# Autodesk Inventor assembly: BUMP_000_Bumpers
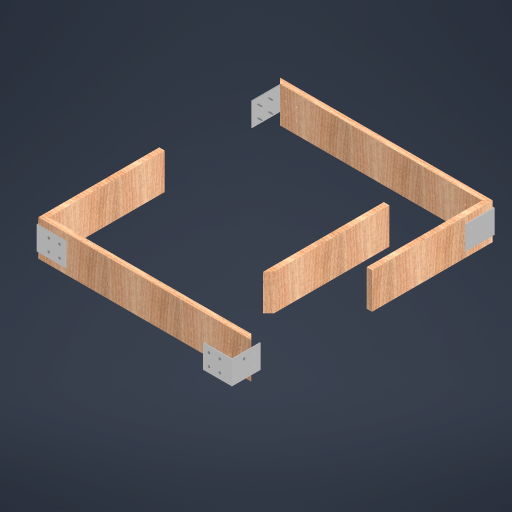
[picture p0: Inventor's stored thumbnail of the model, 512x512]
Saved by Autodesk Inventor 2024.2 (Build 282272000, 272)
## iProperties
Created: 2024-08-06
Part Number: BUMP_000_Bumpers
Document SubType Name: Assembly
Designer: Bryan
Author: Bryan
## Documents named in this file (5)
- C:\Users\bobsb\OneDrive\Documents\GitHub\1622-2024-Summer-CAD-A-Thon\Bumper\BUMP_000_Bumpers.iam
- C:\Users\bobsb\OneDrive\Documents\GitHub\1622-2024-Summer-CAD-A-Thon\Bumper\BUMP_001_Wood1.ipt
- C:\Users\bobsb\OneDrive\Documents\GitHub\1622-2024-Summer-CAD-A-Thon\Bumper\BUMP_002_Wood2.ipt
- C:\Users\bobsb\OneDrive\Documents\GitHub\1622-2024-Summer-CAD-A-Thon\COTS Library\Stucture\COTS_88805K219_Architectural 6063 Aluminum 90 Degree Angle.ipt
- C:\Users\bobsb\OneDrive\Documents\GitHub\1622-2024-Summer-CAD-A-Thon\COTS Library\Fasteners\Wood Screws\COTS_BumperWoodScrew_90031A197_Phillips Flat Head Screws for Wood.ipt
## Components (30 placed, 4 different names)
1. BUMP_001_Wood1:1 — Mate:5, Mate:6, Flush:3, Mate:12, Mate:13
2. BUMP_002_Wood2:1 — Flush:2, Mate:5, Mate:6, Flush:3, Mate:14
3. BUMP_001_Wood1:2 — Mate:1, Flush:1, Mate:2, Flush:2, Mate:7, Mate:9, Mate:27
4. BUMP_002_Wood2:2 — Mate:1, Flush:1, Mate:2, Mate:8
5. COTS_88805K219_Architectural 6063 Aluminum 90 Degree Angle:1 — Mate:7, Mate:8, Mate:19, Mate:20, Mate:21, Mate:22
6. COTS_88805K219_Architectural 6063 Aluminum 90 Degree Angle:2 — Mate:9, Mate:23, Mate:24, Mate:25, Mate:26
7. COTS_88805K219_Architectural 6063 Aluminum 90 Degree Angle:3 — Mate:13, Mate:14
8. COTS_88805K219_Architectural 6063 Aluminum 90 Degree Angle:4 — Mate:12, Mate:15, Mate:16, Mate:17, Mate:18
9. COTS_BumperWoodScrew_90031A197_Phillips Flat Head Screws for Wood:21 — Mate:25, Mate:26
10. BUMP_002_Wood2:3
11. COTS_BumperWoodScrew_90031A197_Phillips Flat Head Screws for Wood:1 — Mate:15, Mate:16
12. COTS_BumperWoodScrew_90031A197_Phillips Flat Head Screws for Wood:2
13. COTS_BumperWoodScrew_90031A197_Phillips Flat Head Screws for Wood:3
14. COTS_BumperWoodScrew_90031A197_Phillips Flat Head Screws for Wood:4
15. COTS_BumperWoodScrew_90031A197_Phillips Flat Head Screws for Wood:5 — Mate:17, Mate:18
16. COTS_BumperWoodScrew_90031A197_Phillips Flat Head Screws for Wood:6
17. COTS_BumperWoodScrew_90031A197_Phillips Flat Head Screws for Wood:7
18. COTS_BumperWoodScrew_90031A197_Phillips Flat Head Screws for Wood:8
19. COTS_BumperWoodScrew_90031A197_Phillips Flat Head Screws for Wood:9 — Mate:19, Mate:20
20. COTS_BumperWoodScrew_90031A197_Phillips Flat Head Screws for Wood:10
21. COTS_BumperWoodScrew_90031A197_Phillips Flat Head Screws for Wood:11
22. COTS_BumperWoodScrew_90031A197_Phillips Flat Head Screws for Wood:12
23. COTS_BumperWoodScrew_90031A197_Phillips Flat Head Screws for Wood:13 — Mate:21, Mate:22
24. COTS_BumperWoodScrew_90031A197_Phillips Flat Head Screws for Wood:14
25. COTS_BumperWoodScrew_90031A197_Phillips Flat Head Screws for Wood:15
26. COTS_BumperWoodScrew_90031A197_Phillips Flat Head Screws for Wood:16
27. COTS_BumperWoodScrew_90031A197_Phillips Flat Head Screws for Wood:17 — Mate:23, Mate:24
28. COTS_BumperWoodScrew_90031A197_Phillips Flat Head Screws for Wood:18
29. COTS_BumperWoodScrew_90031A197_Phillips Flat Head Screws for Wood:19 — Mate:27
30. COTS_BumperWoodScrew_90031A197_Phillips Flat Head Screws for Wood:20
## Component patterns: (4 elements, first: COTS_BumperWoodScrew_90031A197_Phillips Flat Head Screws for Wood:1), (4 elements, first: COTS_BumperWoodScrew_90031A197_Phillips Flat Head Screws for Wood:5), (4 elements, first: COTS_BumperWoodScrew_90031A197_Phillips Flat Head Screws for Wood:9), (4 elements, first: COTS_BumperWoodScrew_90031A197_Phillips Flat Head Screws for Wood:13), (4 elements, first: COTS_BumperWoodScrew_90031A197_Phillips Flat Head Screws for Wood:17)
## Relationships (26: Mate 23, Flush 3)
- Mate:1: BUMP_001_Wood1:2 ↔ BUMP_002_Wood2:2
- Flush:1: BUMP_001_Wood1:2 ↔ BUMP_002_Wood2:2
- Mate:2: BUMP_001_Wood1:2 ↔ BUMP_002_Wood2:2
- Flush:2: BUMP_002_Wood2:1 ↔ BUMP_001_Wood1:2
- Mate:5: BUMP_001_Wood1:1 ↔ BUMP_002_Wood2:1
- Mate:6: BUMP_001_Wood1:1 ↔ BUMP_002_Wood2:1
- Flush:3: BUMP_001_Wood1:1 ↔ BUMP_002_Wood2:1
- Mate:7: BUMP_001_Wood1:2 ↔ COTS_88805K219_Architectural 6063 Aluminum 90 Degree Angle:1
- Mate:8: BUMP_002_Wood2:2 ↔ COTS_88805K219_Architectural 6063 Aluminum 90 Degree Angle:1
- Mate:9: BUMP_001_Wood1:2 ↔ COTS_88805K219_Architectural 6063 Aluminum 90 Degree Angle:2
- Mate:12: BUMP_001_Wood1:1 ↔ COTS_88805K219_Architectural 6063 Aluminum 90 Degree Angle:4
- Mate:13: BUMP_001_Wood1:1 ↔ COTS_88805K219_Architectural 6063 Aluminum 90 Degree Angle:3
- Mate:14: BUMP_002_Wood2:1 ↔ COTS_88805K219_Architectural 6063 Aluminum 90 Degree Angle:3
- Mate:15: COTS_88805K219_Architectural 6063 Aluminum 90 Degree Angle:4 ↔ COTS_BumperWoodScrew_90031A197_Phillips Flat Head Screws for Wood:1
- Mate:16: COTS_88805K219_Architectural 6063 Aluminum 90 Degree Angle:4 ↔ COTS_BumperWoodScrew_90031A197_Phillips Flat Head Screws for Wood:1
- Mate:17: COTS_88805K219_Architectural 6063 Aluminum 90 Degree Angle:4 ↔ COTS_BumperWoodScrew_90031A197_Phillips Flat Head Screws for Wood:5
- Mate:18: COTS_88805K219_Architectural 6063 Aluminum 90 Degree Angle:4 ↔ COTS_BumperWoodScrew_90031A197_Phillips Flat Head Screws for Wood:5
- Mate:19: COTS_88805K219_Architectural 6063 Aluminum 90 Degree Angle:1 ↔ COTS_BumperWoodScrew_90031A197_Phillips Flat Head Screws for Wood:9
- Mate:20: COTS_88805K219_Architectural 6063 Aluminum 90 Degree Angle:1 ↔ COTS_BumperWoodScrew_90031A197_Phillips Flat Head Screws for Wood:9
- Mate:21: COTS_88805K219_Architectural 6063 Aluminum 90 Degree Angle:1 ↔ COTS_BumperWoodScrew_90031A197_Phillips Flat Head Screws for Wood:13
- Mate:22: COTS_88805K219_Architectural 6063 Aluminum 90 Degree Angle:1 ↔ COTS_BumperWoodScrew_90031A197_Phillips Flat Head Screws for Wood:13
- Mate:23: COTS_88805K219_Architectural 6063 Aluminum 90 Degree Angle:2 ↔ COTS_BumperWoodScrew_90031A197_Phillips Flat Head Screws for Wood:17
- Mate:24: COTS_88805K219_Architectural 6063 Aluminum 90 Degree Angle:2 ↔ COTS_BumperWoodScrew_90031A197_Phillips Flat Head Screws for Wood:17
- Mate:25: COTS_88805K219_Architectural 6063 Aluminum 90 Degree Angle:2 ↔ COTS_BumperWoodScrew_90031A197_Phillips Flat Head Screws for Wood:21
- Mate:26: COTS_88805K219_Architectural 6063 Aluminum 90 Degree Angle:2 ↔ COTS_BumperWoodScrew_90031A197_Phillips Flat Head Screws for Wood:21
- Mate:27: BUMP_001_Wood1:2 ↔ COTS_BumperWoodScrew_90031A197_Phillips Flat Head Screws for Wood:19
